# Autodesk Inventor assembly: Assembly5
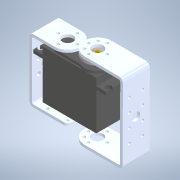
[picture p0: Inventor's stored thumbnail of the model, 180x180]
Saved by Autodesk Inventor 2022 (Build 260153000, 153)
## iProperties
Created: 2022-04-22
Part Number: Assembly5
Document SubType Name: Assembly
Designer: HP
Author: HP
## Documents named in this file (5)
- C:\Users\HP\Documents\Inventor\spider\Assembly5.iam
- C:\Users\HP\Downloads\tower-pro-mg996r-servo-1.snapshot.3\Tower Pro MG996R.ipt
- C:\Users\HP\Downloads\Servo horn v2.ipt
- C:\Users\HP\Downloads\demir1.ipt
- C:\Users\HP\Downloads\demir2.ipt
## Components (4 placed, 4 different names)
1. Tower Pro MG996R:1 — Flush:1, Mate:1, Flush:2, Mate:4
2. Servo horn v2:1 — Flush:1, Mate:2, Mate:3, Rotational:1, Rotational:2
3. demir1:1 — Mate:2, Mate:3, Rotational:1, Rotational:2
4. demir2:1 — Mate:1, Flush:2, Mate:4
## Relationships (8: Mate 4, Flush 2, RevoluteJoint 2)
- Flush:1: Tower Pro MG996R:1 ↔ Servo horn v2:1
- Mate:1: Tower Pro MG996R:1 ↔ demir2:1
- Flush:2: Tower Pro MG996R:1 ↔ demir2:1
- Mate:2: Servo horn v2:1 ↔ demir1:1
- Mate:3: Servo horn v2:1 ↔ demir1:1
- Mate:4 (1.27 mm): Tower Pro MG996R:1 ↔ demir2:1
- Rotational:1 [RevoluteJoint]: Servo horn v2:1 ↔ demir1:1
- Rotational:2 [RevoluteJoint]: Servo horn v2:1 ↔ demir1:1
